# Autodesk Inventor assembly: SAR330 + fixed coupler2 front
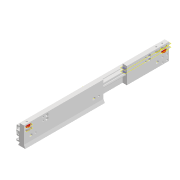
[picture p0: Inventor's stored thumbnail of the model, 180x180]
Saved by Autodesk Inventor 2020 (Build 240168000, 168)
## iProperties
Created: 2019-11-17
Part Number: SAR330 + fixed coupler2 front
Document SubType Name: Assembly
Designer: ball
Author: ball
## Documents named in this file (5)
- C:\FTC\FTC8863CAD\2019 Robot\Delivery\SAR330 + fixed couplers front.iam
- C:\FTC\FTC8863CAD\Misumi\SAR330\SAR330 440 offset.iam
- C:\FTC\FTC8863CAD\2019 Robot\Delivery\Coupler bottom fixed + pulleys.iam
- C:\FTC\FTC8863CAD\2019 Robot\Delivery\Coupler top fixed front + pulleys.iam
- C:\FTC\FTC8863CAD\Actobotics\634 parts\634266.ipt
## Components (4 placed, 4 different names)
1. SAR330 440 offset:1 [sub-assembly] — Mate:1, Mate:2, Angle:1, Mate:3, Mate:4, Angle:2
2. Coupler bottom fixed + pulleys:1 [sub-assembly] — Mate:1, Mate:2, Angle:1, Mate:5, Mate:6
3. Coupler top fixed front + pulleys:1 [sub-assembly] — Mate:3, Mate:4, Angle:2
4. 634266:1 — Mate:5, Mate:6
## Relationships (8: Mate 6, Angle 2)
- Mate:1: SAR330 440 offset:1 ↔ Coupler bottom fixed + pulleys:1
- Mate:2: SAR330 440 offset:1 ↔ Coupler bottom fixed + pulleys:1
- Angle:1 (0 deg): SAR330 440 offset:1 ↔ Coupler bottom fixed + pulleys:1
- Mate:3: SAR330 440 offset:1 ↔ Coupler top fixed front + pulleys:1
- Mate:4: SAR330 440 offset:1 ↔ Coupler top fixed front + pulleys:1
- Angle:2 (0 deg): SAR330 440 offset:1 ↔ Coupler top fixed front + pulleys:1
- Mate:5: Coupler bottom fixed + pulleys:1 ↔ 634266:1
- Mate:6: Coupler bottom fixed + pulleys:1 ↔ 634266:1
